# Autodesk Inventor assembly: Busbar Assembly
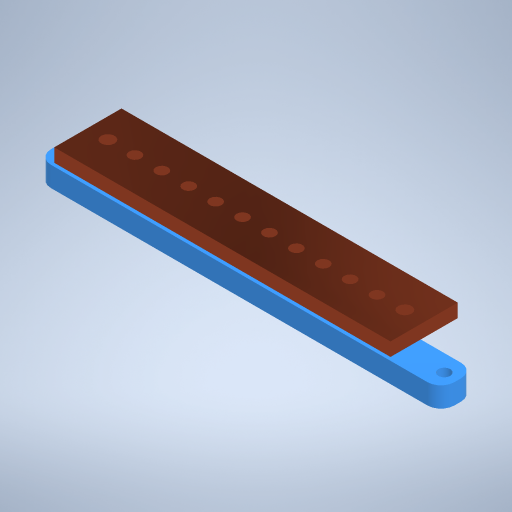
[picture p0: Inventor's stored thumbnail of the model, 512x512]
Saved by Autodesk Inventor 2023 (Build 270158000, 158)
## iProperties
Created: 2023-03-08
Part Number: Busbar Assembly
Document SubType Name: Assembly
Designer: cheng
Author: cheng
## Documents named in this file (3)
- C:\Users\cheng\Desktop\4th Year Project\Inventor\16 th Assembly\Busbar\Busbar Assembly.iam
- C:\Users\cheng\Desktop\4th Year Project\Inventor\16 th Assembly\Busbar\Busbar Base.ipt
- C:\Users\cheng\Desktop\4th Year Project\Inventor\16 th Assembly\Busbar\Busbar Copper.ipt
## Components (2 placed, 2 different names)
1. Busbar Base:1 — Mate:1, Mate:2, Mate:3
2. Busbar Copper:1 — Mate:1, Mate:2, Mate:3
## Relationships (3: Mate 3)
- Mate:1: Busbar Base:1 ↔ Busbar Copper:1
- Mate:2: Busbar Base:1 ↔ Busbar Copper:1
- Mate:3: Busbar Base:1 ↔ Busbar Copper:1
